# Autodesk Inventor assembly: aircilinder_45
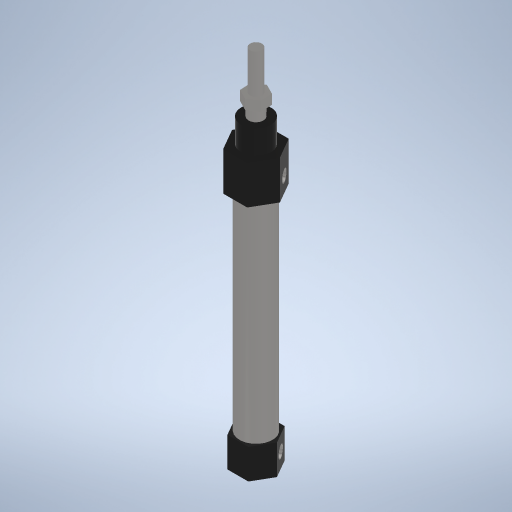
[picture p0: Inventor's stored thumbnail of the model, 512x512]
Saved by Autodesk Inventor 2024 (Build 280153020, 153B)
## iProperties
Created: 2023-10-04
Part Number: aircilinder_45
Document SubType Name: Assembly
Designer: haruy
Author: haruy
## Documents named in this file (3)
- C:\Users\ryogo\OneDrive - Kyushu University\KURT_工房共有\2023~2024\ハード\CAD\2024NHK\000_parts\エアシリンダー\airclinder\aircilinder_45.iam
- C:\Users\ryogo\OneDrive - Kyushu University\KURT_工房共有\2023~2024\ハード\CAD\2024NHK\000_parts\エアシリンダー\airclinder\S5_65_AIR_SA.ipt
- C:\Users\ryogo\OneDrive - Kyushu University\KURT_工房共有\2023~2024\ハード\CAD\2024NHK\000_parts\エアシリンダー\airclinder\S10_90_AIR_SA.ipt
## Components (2 placed, 2 different names)
1. S5_65_AIR_SA:1 — 円柱状:1
2. S10_90_AIR_SA:1 — 円柱状:1
## Relationships (1: CylindricalJoint 1)
- 円柱状:1 [CylindricalJoint]: S5_65_AIR_SA:1 ↔ S10_90_AIR_SA:1
